# Autodesk Inventor assembly: pneumatics thing 2
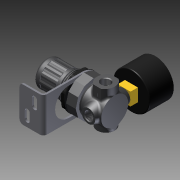
[picture p0: Inventor's stored thumbnail of the model, 180x180]
Saved by Autodesk Inventor 2014 SP1 (Build 180222100, 222)
## iProperties
Created: 2013-12-13
Part Number: pneumatics thing 2
Document SubType Name: Assembly
Designer: Moses
Mass: 1240.84 g
Surface Area: 3277.63 cm^2
Volume: 609.67 cm^3
Density: 2.03527 g/cm^3
Author: Moses
## Documents named in this file (5)
- C:\Users\Arpan\Documents\GitHub\2014buildCAD\pneumatics board\pneumatics thing 2.iam
- C:\Users\Arpan\Documents\GitHub\2014buildCAD\pneumatics board\Pneumatics_Norgren_R07-100-RNEA.ipt
- C:\Users\Arpan\Documents\GitHub\2014buildCAD\pneumatics board\Pneumatics_WIKA_9690242.ipt
- C:\Users\Arpan\Documents\GitHub\2014buildCAD\pneumatics board\Pneumatics_Norgren_18-025-003_Bracket.ipt
- C:\Users\Arpan\Documents\GitHub\2014buildCAD\pneumatics board\Pneumatics_Norgren_18-025-003_Panel Nut.ipt
## Components (4 placed, 4 different names)
1. Pneumatics_Norgren_18-025-003_Bracket:1 — Mate:9, Mate:10, Mate:20
2. Pneumatics_Norgren_R07-100-RNEA:1 — Mate:9, Mate:10, Insert:9, Mate:19
3. Pneumatics_WIKA_9690242:2 — Insert:9
4. Pneumatics_Norgren_18-025-003_Panel Nut:1 — Mate:19, Mate:20
## Relationships (5: Mate 4, Insert 1)
- Mate:9: Pneumatics_Norgren_18-025-003_Bracket:1 ↔ Pneumatics_Norgren_R07-100-RNEA:1
- Mate:10: Pneumatics_Norgren_18-025-003_Bracket:1 ↔ Pneumatics_Norgren_R07-100-RNEA:1
- Insert:9 (1.27 mm): Pneumatics_Norgren_R07-100-RNEA:1 ↔ Pneumatics_WIKA_9690242:2
- Mate:19: Pneumatics_Norgren_R07-100-RNEA:1 ↔ Pneumatics_Norgren_18-025-003_Panel Nut:1
- Mate:20: Pneumatics_Norgren_18-025-003_Bracket:1 ↔ Pneumatics_Norgren_18-025-003_Panel Nut:1
